# Autodesk Inventor assembly: PodSubassembly
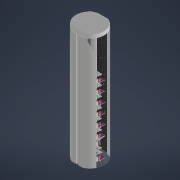
[picture p0: Inventor's stored thumbnail of the model, 180x180]
Saved by Autodesk Inventor 2021 (Build 250183000, 183)
## iProperties
Created: 2021-01-31
Part Number: PodSubassembly
Document SubType Name: Assembly
Designer: argon
Author: argon
## Documents named in this file (6)
- C:\Users\argon\OneDrive\Documents\GrabCAD\EngOne Maroons\Pod Subassembly\PodSubassembly.iam
- C:\Users\argon\OneDrive\Documents\GrabCAD\EngOne Maroons\Pod Subassembly\PodShell.ipt
- C:\Users\argon\OneDrive\Documents\GrabCAD\EngOne Maroons\Pod Subassembly\PodFloorSubAssembly.iam
- C:\Users\argon\OneDrive\Documents\GrabCAD\EngOne Maroons\Ceiling Subassembly\DarkCeilingSubassembly.iam
- C:\Users\argon\OneDrive\Documents\GrabCAD\EngOne Maroons\Luggage Subassembly\LuggageSubassembly.iam
- C:\Users\argon\OneDrive\Documents\GrabCAD\EngOne Maroons\Luggage Subassembly\SlopeFloor.ipt
## Components (5 placed, 5 different names)
1. PodShell:1 — Mate:1, Mate:2, Mate:3, Mate:4, Flush:2, Mate:5, Mate:6, Flush:3
2. PodFloorSubAssembly:1 [sub-assembly] — Mate:1, Mate:2, Flush:3, Mate:7, Mate:8, Mate:9
3. DarkCeilingSubassembly:1 [sub-assembly] — Mate:3, Mate:4, Flush:2, Angle:1
4. LuggageSubassembly:1 [sub-assembly] — Mate:5, Mate:6, Angle:1
5. SlopeFloor:1 — Mate:7, Mate:8, Mate:9
## Relationships (12: Mate 9, Flush 2, Angle 1)
- Mate:1: PodShell:1 ↔ PodFloorSubAssembly:1
- Mate:2: PodShell:1 ↔ PodFloorSubAssembly:1
- Mate:3: PodShell:1 ↔ DarkCeilingSubassembly:1
- Mate:4: PodShell:1 ↔ DarkCeilingSubassembly:1
- Flush:2: PodShell:1 ↔ DarkCeilingSubassembly:1
- Mate:5: PodShell:1 ↔ LuggageSubassembly:1
- Mate:6: PodShell:1 ↔ LuggageSubassembly:1
- Flush:3: PodShell:1 ↔ PodFloorSubAssembly:1
- Mate:7: PodFloorSubAssembly:1 ↔ SlopeFloor:1
- Mate:8: PodFloorSubAssembly:1 ↔ SlopeFloor:1
- Mate:9: PodFloorSubAssembly:1 ↔ SlopeFloor:1
- Angle:1 (0 deg): DarkCeilingSubassembly:1 ↔ LuggageSubassembly:1
